# Autodesk Inventor assembly: KND-2610 Main way 01
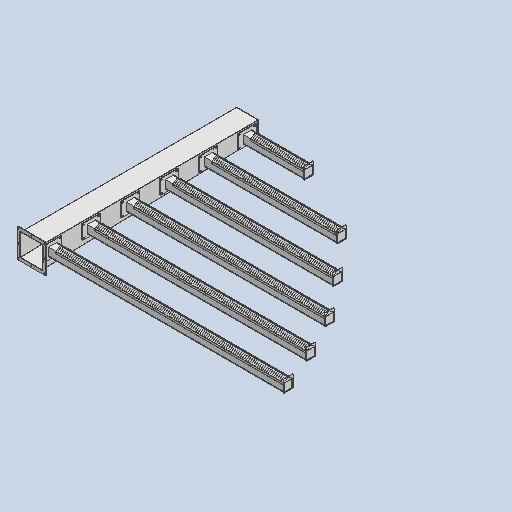
[picture p0: Inventor's stored thumbnail of the model, 512x512]
Saved by Autodesk Inventor 2026.2 (Build 302298000, 298)
## iProperties
Created: 2026-05-12
Part Number: KND-2610 Main way 01
Document SubType Name: Assembly
Designer: admin
Author: admin
## Documents named in this file (19)
- C:\Users\admin\Documents\Inventor\KND-DistribSystem\DRS_D1200\KND-2610 Main way 01.iam
- C:\Users\admin\Documents\Inventor\KND-DistribSystem\DRS_D1200\KND-1425 DrSysB Way FLANGE 01.ipt
- C:\Users\admin\Documents\Inventor\KND-DistribSystem\DRS_D1200\KND-1663 DrSysB way tube 4 01.ipt
- C:\Users\admin\Documents\Inventor\KND-DistribSystem\DRS_D1200\KND-1662 DrSysB way tube 2 01.ipt
- C:\Users\admin\Documents\Inventor\KND-DistribSystem\DRS_D1200\KND-1666 FDS 1000 CUP 1 01.ipt
- C:\Users\admin\Documents\Inventor\KND-DistribSystem\DRS_D1200\KND-1422 DrSysB diameter way up 01.ipt
- C:\Users\admin\Documents\Inventor\KND-DistribSystem\DRS_D1200\KND-1423 DrSysB diameter way down 01.ipt
- C:\Users\admin\Documents\Inventor\KND-DistribSystem\DRS_D1200\KND-1424 DrSysB diam way cup 01.ipt
- C:\Users\admin\Documents\Inventor\KND-DistribSystem\DRS_D1200\KND-1661 DrSysB way tube 1 01.ipt
- C:\Users\admin\Documents\Inventor\KND-DistribSystem\DRS_D1200\KND-5311 DrSysB roof 1 01.ipt
- C:\Users\admin\Documents\Inventor\KND-DistribSystem\DRS_D1200\KND-5321 DrSysB roof 2 01.ipt
- C:\Users\admin\Documents\Inventor\KND-DistribSystem\DRS_D1200\KND-5333 DrSysB roof 3 01.ipt
- C:\Users\admin\Documents\Inventor\KND-DistribSystem\DRS_D1200\KND-1664 DrSysB way tube 44 01.ipt
- C:\Users\admin\Documents\Inventor\KND-DistribSystem\DRS_D1200\KND-5335 DrSysB roof 33 01.ipt
- C:\Users\admin\Documents\Inventor\KND-DistribSystem\DRS_D1200\KND-1667 DrSysB way tube 5 01.ipt
- C:\Users\admin\Documents\Inventor\KND-DistribSystem\DRS_D1200\KND-5337 DrSysB roof 5 01.ipt
- C:\Users\admin\Documents\Inventor\KND-DistribSystem\DRS_D1200\KND-1668 DrSysB way tube 6 01.ipt
- C:\Users\admin\Documents\Inventor\KND-DistribSystem\DRS_D1200\KND-5338 DrSysB roof 6 01.ipt
- C:\Users\admin\Documents\Inventor\KND-DistribSystem\DRS_D1200\KND-1426 DrSysB Main way FLANGE 01.ipt
## Components (28 placed, 20 different names)
1. PRS 1425 DrSysB Way FLANGE_D1200:1 — Mate:34, Mate:40, Mate:41
2. PRS 1662 DrSysB way tube 4_D1200:1 — Mate:55, Mate:56, Mate:57, Mate:80, Mate:81, Flush:34, Mate:99, Mate:100, Mate:111, Flush:48, Flush:49
3. PRS 1662 DrSysB way tube 2_D1200:1 — Mate:52, Mate:53, Mate:54, Mate:78, Mate:79, Flush:33, Mate:97, Mate:98, Mate:110, Flush:46, Flush:47
4. PRS-1666 FDS 1000 CUP 1_D1200:1 — Mate:109, Flush:44, Flush:45
5. PRS 1422 DrSysB diameter way up_D1200:1 — Flush:10, Flush:9, Mate:11, Rigid:23, Mate:108
6. PRS 1423 DrSysB diameter way down_D1200:1 — Rigid:23, Mate:16, Mate:17, Mate:18, Mate:34, Mate:52, Mate:53, Mate:54, Mate:55, Mate:56, Mate:57, Mate:58, Mate:59, Mate:60, Mate:61, Mate:62, Mate:63, Mate:64, Mate:65, Mate:66, Mate:69, Mate:71, Mate:73, Mate:75, Mate:77, Mate:107, Flush:43
7. PRS 1424 DrSysB diam way cup_D1200:1 — Flush:10, Flush:9, Mate:11
8. PRS 1425 DrSysB Way FLANGE_D1200:2 — Mate:69, Mate:78, Mate:79
9. PRS 1425 DrSysB Way FLANGE_D1200:3 — Mate:71, Mate:80, Mate:81
10. PRS 1661 DrSysB way tube 1_D1200:1 — Mate:16, Mate:17, Mate:18, Mate:40, Mate:41, Flush:32, Mate:95, Mate:96, Mate:109, Flush:44, Flush:45
11. PRS 5311 DrSysB roof 1_D1200:1 — Flush:32, Mate:95, Mate:96
12. PRS 5321 DrSysB roof 2_D1200:1 — Flush:33, Mate:97, Mate:98
13. PRS 5333 DrSysB roof 3_D1200:1 — Flush:34, Mate:99, Mate:100
14. PRS 1662 DrSysB way tube 44_D1200:1 — Mate:58, Mate:59, Mate:60, Mate:82, Mate:83, Flush:35, Mate:101, Mate:102, Mate:112, Flush:50, Flush:51
15. PRS 5335 DrSysB roof 33_D1200:1 — Flush:35, Mate:101, Mate:102
16. PRS 1425 DrSysB Way FLANGE_D1200:7 — Mate:73, Mate:82, Mate:83
17. KND-1667 DrSysB way tube 5 01:1 — Mate:61, Mate:62, Mate:63, Mate:84, Mate:85, Flush:36, Mate:103, Mate:104, Mate:113, Flush:52, Flush:53
18. KND-5337 DrSysB roof 5 01:1 — Flush:36, Mate:103, Mate:104
19. KND-1425 DrSysB Way FLANGE 01:8 — Mate:75, Mate:84, Mate:85
20. KND-1668 DrSysB way tube 6 01:1 — Mate:64, Mate:65, Mate:66, Mate:86, Mate:87, Flush:37, Mate:105, Mate:106, Mate:114, Flush:54, Flush:55
21. KND-5338 DrSysB roof 6 01:1 — Flush:37, Mate:105, Mate:106
22. KND-1425 DrSysB Way FLANGE 01:9 — Mate:77, Mate:86, Mate:87
23. KND-1666 FDS 1000 CUP 1 01:2 — Mate:110, Flush:46, Flush:47
24. KND-1666 FDS 1000 CUP 1 01:3 — Mate:111, Flush:48, Flush:49
25. KND-1666 FDS 1000 CUP 1 01:4 — Mate:112, Flush:50, Flush:51
26. KND-1666 FDS 1000 CUP 1 01:5 — Mate:113, Flush:52, Flush:53
27. KND-1666 FDS 1000 CUP 1 01:6 — Mate:114, Flush:54, Flush:55
28. KND-1426 DrSysB Main way FLANGE 01:1 — Mate:107, Mate:108, Flush:43
## Relationships (79: Mate 57, Flush 21, WeldJoint 1)
- Flush:10 (1 mm): PRS 1422 DrSysB diameter way up_D1200:1 ↔ PRS 1424 DrSysB diam way cup_D1200:1
- Flush:9 (-1 mm): PRS 1422 DrSysB diameter way up_D1200:1 ↔ PRS 1424 DrSysB diam way cup_D1200:1
- Mate:11: PRS 1422 DrSysB diameter way up_D1200:1 ↔ PRS 1424 DrSysB diam way cup_D1200:1
- Rigid:23 [WeldJoint]: PRS 1422 DrSysB diameter way up_D1200:1 ↔ PRS 1423 DrSysB diameter way down_D1200:1
- Mate:16: PRS 1423 DrSysB diameter way down_D1200:1 ↔ PRS 1661 DrSysB way tube 1_D1200:1
- Mate:17 (0.25 mm): PRS 1423 DrSysB diameter way down_D1200:1 ↔ PRS 1661 DrSysB way tube 1_D1200:1
- Mate:18 (0.25 mm): PRS 1423 DrSysB diameter way down_D1200:1 ↔ PRS 1661 DrSysB way tube 1_D1200:1
- Mate:34: PRS 1425 DrSysB Way FLANGE_D1200:1 ↔ PRS 1423 DrSysB diameter way down_D1200:1
- Mate:40 (0.1 mm): PRS 1425 DrSysB Way FLANGE_D1200:1 ↔ PRS 1661 DrSysB way tube 1_D1200:1
- Mate:41 (0.1 mm): PRS 1425 DrSysB Way FLANGE_D1200:1 ↔ PRS 1661 DrSysB way tube 1_D1200:1
- Mate:52: PRS 1662 DrSysB way tube 2_D1200:1 ↔ PRS 1423 DrSysB diameter way down_D1200:1
- Mate:53 (0.25 mm): PRS 1662 DrSysB way tube 2_D1200:1 ↔ PRS 1423 DrSysB diameter way down_D1200:1
- Mate:54 (0.25 mm): PRS 1662 DrSysB way tube 2_D1200:1 ↔ PRS 1423 DrSysB diameter way down_D1200:1
- Mate:55: PRS 1662 DrSysB way tube 4_D1200:1 ↔ PRS 1423 DrSysB diameter way down_D1200:1
- Mate:56 (0.25 mm): PRS 1662 DrSysB way tube 4_D1200:1 ↔ PRS 1423 DrSysB diameter way down_D1200:1
- Mate:57 (0.25 mm): PRS 1662 DrSysB way tube 4_D1200:1 ↔ PRS 1423 DrSysB diameter way down_D1200:1
- Mate:58: PRS 1423 DrSysB diameter way down_D1200:1 ↔ PRS 1662 DrSysB way tube 44_D1200:1
- Mate:59 (0.25 mm): PRS 1423 DrSysB diameter way down_D1200:1 ↔ PRS 1662 DrSysB way tube 44_D1200:1
- Mate:60 (0.25 mm): PRS 1423 DrSysB diameter way down_D1200:1 ↔ PRS 1662 DrSysB way tube 44_D1200:1
- Mate:61: PRS 1423 DrSysB diameter way down_D1200:1 ↔ KND-1667 DrSysB way tube 5 01:1
- Mate:62 (0.25 mm): PRS 1423 DrSysB diameter way down_D1200:1 ↔ KND-1667 DrSysB way tube 5 01:1
- Mate:63 (0.25 mm): PRS 1423 DrSysB diameter way down_D1200:1 ↔ KND-1667 DrSysB way tube 5 01:1
- Mate:64: PRS 1423 DrSysB diameter way down_D1200:1 ↔ KND-1668 DrSysB way tube 6 01:1
- Mate:65 (0.25 mm): PRS 1423 DrSysB diameter way down_D1200:1 ↔ KND-1668 DrSysB way tube 6 01:1
- Mate:66 (0.25 mm): PRS 1423 DrSysB diameter way down_D1200:1 ↔ KND-1668 DrSysB way tube 6 01:1
- Mate:69: PRS 1423 DrSysB diameter way down_D1200:1 ↔ PRS 1425 DrSysB Way FLANGE_D1200:2
- Mate:71: PRS 1423 DrSysB diameter way down_D1200:1 ↔ PRS 1425 DrSysB Way FLANGE_D1200:3
- Mate:73: PRS 1423 DrSysB diameter way down_D1200:1 ↔ PRS 1425 DrSysB Way FLANGE_D1200:7
- Mate:75: PRS 1423 DrSysB diameter way down_D1200:1 ↔ KND-1425 DrSysB Way FLANGE 01:8
- Mate:77: PRS 1423 DrSysB diameter way down_D1200:1 ↔ KND-1425 DrSysB Way FLANGE 01:9
- Mate:78 (0.1 mm): PRS 1662 DrSysB way tube 2_D1200:1 ↔ PRS 1425 DrSysB Way FLANGE_D1200:2
- Mate:79 (0.1 mm): PRS 1662 DrSysB way tube 2_D1200:1 ↔ PRS 1425 DrSysB Way FLANGE_D1200:2
- Mate:80 (0.1 mm): PRS 1662 DrSysB way tube 4_D1200:1 ↔ PRS 1425 DrSysB Way FLANGE_D1200:3
- Mate:81 (0.1 mm): PRS 1662 DrSysB way tube 4_D1200:1 ↔ PRS 1425 DrSysB Way FLANGE_D1200:3
- Mate:82 (0.1 mm): PRS 1662 DrSysB way tube 44_D1200:1 ↔ PRS 1425 DrSysB Way FLANGE_D1200:7
- Mate:83 (0.1 mm): PRS 1662 DrSysB way tube 44_D1200:1 ↔ PRS 1425 DrSysB Way FLANGE_D1200:7
- Mate:84 (0.1 mm): KND-1667 DrSysB way tube 5 01:1 ↔ KND-1425 DrSysB Way FLANGE 01:8
- Mate:85 (0.1 mm): KND-1667 DrSysB way tube 5 01:1 ↔ KND-1425 DrSysB Way FLANGE 01:8
- Mate:86 (0.1 mm): KND-1668 DrSysB way tube 6 01:1 ↔ KND-1425 DrSysB Way FLANGE 01:9
- Mate:87 (0.1 mm): KND-1668 DrSysB way tube 6 01:1 ↔ KND-1425 DrSysB Way FLANGE 01:9
- Flush:32: PRS 1661 DrSysB way tube 1_D1200:1 ↔ PRS 5311 DrSysB roof 1_D1200:1
- Mate:95 (0.1576 mm): PRS 1661 DrSysB way tube 1_D1200:1 ↔ PRS 5311 DrSysB roof 1_D1200:1
- Mate:96 (-9.5 mm): PRS 1661 DrSysB way tube 1_D1200:1 ↔ PRS 5311 DrSysB roof 1_D1200:1
- Flush:33: PRS 1662 DrSysB way tube 2_D1200:1 ↔ PRS 5321 DrSysB roof 2_D1200:1
- Mate:97 (0.1576 mm): PRS 1662 DrSysB way tube 2_D1200:1 ↔ PRS 5321 DrSysB roof 2_D1200:1
- Mate:98 (-9.5 mm): PRS 1662 DrSysB way tube 2_D1200:1 ↔ PRS 5321 DrSysB roof 2_D1200:1
- Flush:34: PRS 1662 DrSysB way tube 4_D1200:1 ↔ PRS 5333 DrSysB roof 3_D1200:1
- Mate:99 (0.1576 mm): PRS 1662 DrSysB way tube 4_D1200:1 ↔ PRS 5333 DrSysB roof 3_D1200:1
- Mate:100 (-9.5 mm): PRS 1662 DrSysB way tube 4_D1200:1 ↔ PRS 5333 DrSysB roof 3_D1200:1
- Flush:35: PRS 1662 DrSysB way tube 44_D1200:1 ↔ PRS 5335 DrSysB roof 33_D1200:1
- Mate:101 (0.1576 mm): PRS 1662 DrSysB way tube 44_D1200:1 ↔ PRS 5335 DrSysB roof 33_D1200:1
- Mate:102 (-9.5 mm): PRS 1662 DrSysB way tube 44_D1200:1 ↔ PRS 5335 DrSysB roof 33_D1200:1
- Flush:36: KND-1667 DrSysB way tube 5 01:1 ↔ KND-5337 DrSysB roof 5 01:1
- Mate:103 (0.1576 mm): KND-1667 DrSysB way tube 5 01:1 ↔ KND-5337 DrSysB roof 5 01:1
- Mate:104 (-9.5 mm): KND-1667 DrSysB way tube 5 01:1 ↔ KND-5337 DrSysB roof 5 01:1
- Flush:37: KND-1668 DrSysB way tube 6 01:1 ↔ KND-5338 DrSysB roof 6 01:1
- Mate:105 (0.1576 mm): KND-1668 DrSysB way tube 6 01:1 ↔ KND-5338 DrSysB roof 6 01:1
- Mate:106 (-9.5 mm): KND-1668 DrSysB way tube 6 01:1 ↔ KND-5338 DrSysB roof 6 01:1
- Mate:107 (1.1 mm): PRS 1423 DrSysB diameter way down_D1200:1 ↔ KND-1426 DrSysB Main way FLANGE 01:1
- Mate:108 (0.1 mm): PRS 1422 DrSysB diameter way up_D1200:1 ↔ KND-1426 DrSysB Main way FLANGE 01:1
- Flush:43: PRS 1423 DrSysB diameter way down_D1200:1 ↔ KND-1426 DrSysB Main way FLANGE 01:1
- Mate:109: PRS-1666 FDS 1000 CUP 1_D1200:1 ↔ PRS 1661 DrSysB way tube 1_D1200:1
- Flush:44 (-3 mm): PRS-1666 FDS 1000 CUP 1_D1200:1 ↔ PRS 1661 DrSysB way tube 1_D1200:1
- Flush:45 (-2 mm): PRS-1666 FDS 1000 CUP 1_D1200:1 ↔ PRS 1661 DrSysB way tube 1_D1200:1
- Mate:110: PRS 1662 DrSysB way tube 2_D1200:1 ↔ KND-1666 FDS 1000 CUP 1 01:2
- Flush:46 (-3 mm): PRS 1662 DrSysB way tube 2_D1200:1 ↔ KND-1666 FDS 1000 CUP 1 01:2
- Flush:47 (-2 mm): PRS 1662 DrSysB way tube 2_D1200:1 ↔ KND-1666 FDS 1000 CUP 1 01:2
- Mate:111: PRS 1662 DrSysB way tube 4_D1200:1 ↔ KND-1666 FDS 1000 CUP 1 01:3
- Flush:48 (-3 mm): PRS 1662 DrSysB way tube 4_D1200:1 ↔ KND-1666 FDS 1000 CUP 1 01:3
- Flush:49 (-2 mm): PRS 1662 DrSysB way tube 4_D1200:1 ↔ KND-1666 FDS 1000 CUP 1 01:3
- Mate:112: PRS 1662 DrSysB way tube 44_D1200:1 ↔ KND-1666 FDS 1000 CUP 1 01:4
- Flush:50 (-3 mm): PRS 1662 DrSysB way tube 44_D1200:1 ↔ KND-1666 FDS 1000 CUP 1 01:4
- Flush:51 (-2 mm): PRS 1662 DrSysB way tube 44_D1200:1 ↔ KND-1666 FDS 1000 CUP 1 01:4
- Mate:113: KND-1667 DrSysB way tube 5 01:1 ↔ KND-1666 FDS 1000 CUP 1 01:5
- Flush:52 (-3 mm): KND-1667 DrSysB way tube 5 01:1 ↔ KND-1666 FDS 1000 CUP 1 01:5
- Flush:53 (-2 mm): KND-1667 DrSysB way tube 5 01:1 ↔ KND-1666 FDS 1000 CUP 1 01:5
- Mate:114: KND-1668 DrSysB way tube 6 01:1 ↔ KND-1666 FDS 1000 CUP 1 01:6
- Flush:54 (-3 mm): KND-1668 DrSysB way tube 6 01:1 ↔ KND-1666 FDS 1000 CUP 1 01:6
- Flush:55 (-2 mm): KND-1668 DrSysB way tube 6 01:1 ↔ KND-1666 FDS 1000 CUP 1 01:6
